# Autodesk Inventor assembly: still_system
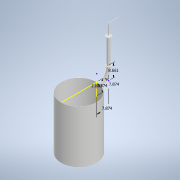
[picture p0: Inventor's stored thumbnail of the model, 180x180]
Saved by Autodesk Inventor 2020 (Build 240168000, 168)
## iProperties
Created: 2022-09-03
Part Number: still_system
Document SubType Name: Assembly
Designer: Intuito_PC
Author: Intuito_PC
## Documents named in this file (4)
- C:\Users\Intuito_PC\Desktop\academ\final_yr_project\auto_distiller\report_work\Project_Implementation_Report\CAD\still_system.iam
- C:\Users\Intuito_PC\Desktop\academ\final_yr_project\auto_distiller\report_work\Project_Implementation_Report\CAD\still.ipt
- C:\Users\Intuito_PC\Desktop\academ\final_yr_project\auto_distiller\report_work\Project_Implementation_Report\CAD\fractionating_column.ipt
- C:\Users\Intuito_PC\Desktop\academ\final_yr_project\auto_distiller\report_work\Project_Implementation_Report\CAD\fractionating_column_cover.ipt
## Components (3 placed, 3 different names)
1. still:1 — Insert:1
2. fractionating_column:1 — Insert:1, Insert:2, Insert:3
3. fractionating_column_cover:1 — Insert:2, Insert:3
## Relationships (3: Insert 3)
- Insert:1: still:1 ↔ fractionating_column:1
- Insert:2: fractionating_column:1 ↔ fractionating_column_cover:1
- Insert:3: fractionating_column:1 ↔ fractionating_column_cover:1
